# Autodesk Inventor assembly: Assembly1
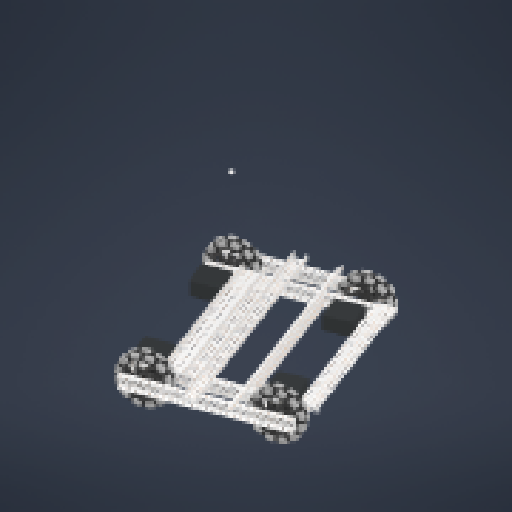
[picture p0: Inventor's stored thumbnail of the model, 512x512]
Saved by Autodesk Inventor 2023 (Build 270158000, 158)
## iProperties
Created: 2022-12-20
Part Number: Assembly1
Document SubType Name: Assembly
Designer: macbook
Author: macbook
## Documents named in this file (8)
- C:\Users\Windows Macbook\Desktop\tank.iam
- C:\Users\Windows Macbook\Documents\Inventor\Content Center Files\VEX-CAD-Inventor-1.4.0\Structure\C Channel\Aluminum 1x2x1\Alu C 1x2x1x25.ipt
- C:\Users\Windows Macbook\Documents\Inventor\Content Center Files\VEX-CAD-Inventor-1.4.0\Electronics\V5 Simple Motor.ipt
- C:\Users\Windows Macbook\Documents\Inventor\Content Center Files\VEX-CAD-Inventor-1.4.0\Motion\Shaft LS\Bearing Flat.ipt
- C:\Users\Windows Macbook\Documents\Inventor\Content Center Files\VEX-CAD-Inventor-1.4.0\Motion\Spacers\Spacer Nylon .313 OD\NSpacer .313 OD x .125.ipt
- C:\Users\macbook\Documents\Inventor\Content Center Files\VEX-CAD-Inventor-1.4.0\Motion\Spacers\Spacer Nylon .313 OD.ipt
- C:\Users\macbook\Documents\Inventor\Content Center Files\VEX-CAD-Inventor-1.4.0\Motion\Wheels\Omni Wheel.iam
- C:\Users\Windows Macbook\Documents\Inventor\Content Center Files\VEX-CAD-Inventor-1.4.0\Motion\Wheels\Omni Wheel\4 Omni, Square.iam
## Components (29 placed, 5 different names)
1. Alu C 1x2x1x25:1 — Insert:2, Insert:42, Insert:43, Insert:44, Insert:45, Insert:46, Insert:47, Insert:48, Insert:49
2. Alu C 1x2x1x25:2 — Insert:1, Insert:27, Insert:28, Insert:29, Insert:30, Insert:36, Insert:37, Insert:38, Insert:39
3. Alu C 1x2x1x25:3 — Insert:1, Insert:2
4. Alu C 1x2x1x25:5 — Insert:31, Insert:32, Insert:40, Insert:41
5. Alu C 1x2x1x25:6 — Insert:65, Insert:66, Insert:67, Insert:68
6. V5 Simple Motor:1 — Insert:44, Insert:45
7. V5 Simple Motor:2 — Insert:42, Insert:43
8. V5 Simple Motor:3 — Insert:36, Insert:37
9. V5 Simple Motor:4 — Insert:27, Insert:28
10. Bearing Flat:2 — Insert:29, Insert:30, Insert:33
11. Bearing Flat:3 — Insert:31, Insert:32, Insert:34
12. NSpacer .313 OD x .125:1 — Insert:33
13. NSpacer .313 OD x .125:2 — Insert:34, Insert:35
14. 4 Omni, Square:1 [sub-assembly] — Insert:35
15. Bearing Flat:4 — Insert:40, Insert:41, Insert:50
16. Bearing Flat:5 — Insert:38, Insert:39, Insert:51
17. Bearing Flat:7 — Insert:48, Insert:49, Insert:71
18. Bearing Flat:9 — Insert:46, Insert:47, Insert:69
19. NSpacer .313 OD x .125:3 — Insert:50, Insert:52
20. NSpacer .313 OD x .125:4 — Insert:51
21. 4 Omni, Square:2 [sub-assembly] — Insert:52
22. Bearing Flat:10 — Insert:65, Insert:66, Insert:70
23. Bearing Flat:11 — Insert:67, Insert:68, Insert:72
24. NSpacer .313 OD x .125:5 — Insert:71
25. NSpacer .313 OD x .125:6
26. NSpacer .313 OD x .125:7 — Insert:69
27. NSpacer .313 OD x .125:8 — Insert:70, Insert:73
28. 4 Omni, Square:3 [sub-assembly] — Insert:72
29. 4 Omni, Square:4 [sub-assembly] — Insert:73
## Relationships (37: Insert 37)
- Insert:1: Alu C 1x2x1x25:2 ↔ Alu C 1x2x1x25:3
- Insert:2: Alu C 1x2x1x25:1 ↔ Alu C 1x2x1x25:3
- Insert:27: Alu C 1x2x1x25:2 ↔ V5 Simple Motor:4
- Insert:28: Alu C 1x2x1x25:2 ↔ V5 Simple Motor:4
- Insert:29: Alu C 1x2x1x25:2 ↔ Bearing Flat:2
- Insert:30: Alu C 1x2x1x25:2 ↔ Bearing Flat:2
- Insert:31: Alu C 1x2x1x25:5 ↔ Bearing Flat:3
- Insert:32: Alu C 1x2x1x25:5 ↔ Bearing Flat:3
- Insert:33: Bearing Flat:2 ↔ NSpacer .313 OD x .125:1
- Insert:34: Bearing Flat:3 ↔ NSpacer .313 OD x .125:2
- Insert:35: NSpacer .313 OD x .125:2 ↔ 4 Omni, Square:1
- Insert:36: Alu C 1x2x1x25:2 ↔ V5 Simple Motor:3
- Insert:37: Alu C 1x2x1x25:2 ↔ V5 Simple Motor:3
- Insert:38: Alu C 1x2x1x25:2 ↔ Bearing Flat:5
- Insert:39: Alu C 1x2x1x25:2 ↔ Bearing Flat:5
- Insert:40: Alu C 1x2x1x25:5 ↔ Bearing Flat:4
- Insert:41: Alu C 1x2x1x25:5 ↔ Bearing Flat:4
- Insert:42: Alu C 1x2x1x25:1 ↔ V5 Simple Motor:2
- Insert:43: Alu C 1x2x1x25:1 ↔ V5 Simple Motor:2
- Insert:44: Alu C 1x2x1x25:1 ↔ V5 Simple Motor:1
- Insert:45: Alu C 1x2x1x25:1 ↔ V5 Simple Motor:1
- Insert:46: Alu C 1x2x1x25:1 ↔ Bearing Flat:9
- Insert:47: Alu C 1x2x1x25:1 ↔ Bearing Flat:9
- Insert:48: Alu C 1x2x1x25:1 ↔ Bearing Flat:7
- Insert:49: Alu C 1x2x1x25:1 ↔ Bearing Flat:7
- Insert:50: Bearing Flat:4 ↔ NSpacer .313 OD x .125:3
- Insert:51: Bearing Flat:5 ↔ NSpacer .313 OD x .125:4
- Insert:52: NSpacer .313 OD x .125:3 ↔ 4 Omni, Square:2
- Insert:65: Alu C 1x2x1x25:6 ↔ Bearing Flat:10
- Insert:66: Alu C 1x2x1x25:6 ↔ Bearing Flat:10
- Insert:67: Alu C 1x2x1x25:6 ↔ Bearing Flat:11
- Insert:68: Alu C 1x2x1x25:6 ↔ Bearing Flat:11
- Insert:69: Bearing Flat:9 ↔ NSpacer .313 OD x .125:7
- Insert:70: Bearing Flat:10 ↔ NSpacer .313 OD x .125:8
- Insert:71: Bearing Flat:7 ↔ NSpacer .313 OD x .125:5
- Insert:72: Bearing Flat:11 ↔ 4 Omni, Square:3
- Insert:73: NSpacer .313 OD x .125:8 ↔ 4 Omni, Square:4
